# Autodesk Inventor assembly: robotModularAutoreconnfigurable
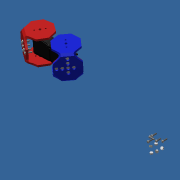
[picture p0: Inventor's stored thumbnail of the model, 180x180]
Saved by Autodesk Inventor 2014 (Build 180170000, 170)
## iProperties
Created: 2014-04-30
Part Number: robotModularAutoreconnfigurable
Document SubType Name: Assembly
Designer: Lefo
Author: Lefo
## Documents named in this file (9)
- C:\Users\Lefo\Documents\Inventor\academy\final project\robotModularAutoreconnfigurable.iam
- C:\Users\Lefo\Documents\Inventor\academy\servo power HD1501MG\servomotorFakeShast.iam
- C:\Users\Lefo\Documents\Inventor\academy\final project\linkoct.ipt
- C:\Users\Lefo\Documents\Inventor\academy\iman.ipt
- C:\Users\Lefo\Documents\Inventor\academy\portatuerca.ipt
- C:\Users\Lefo\Documents\Inventor\academy\final project\linkoctsecundario.ipt
- C:\Users\Lefo\Documents\Inventor\Content Center Files\R2014\en-US\ISO 7045(1)\ISO 7045 - M3 x 12 - 4.8 - HDIN EN ISO.ipt
- C:\Users\Lefo\Documents\Inventor\academy\servo power HD1501MG\acople para eje falso.ipt
- C:\Users\Lefo\Documents\Inventor\Content Center Files\R2014\en-US\ISO 7045(1)\ISO 7045 - M3 x 10 - 4.8 - HDIN EN ISO.ipt
## Components (30 placed, 8 different names)
1. servomotorFakeShast:1 [sub-assembly] — Mate:1, Flush:1, Flush:2, Insert:11, Insert:19
2. servomotorFakeShast:2 [sub-assembly] — Mate:1, Flush:1, Flush:2, Insert:10, Mate:2, Insert:18
3. linkoct:2 — Insert:3, Insert:4, Insert:5, Insert:6, Insert:7, Insert:8, Insert:9, Insert:11, Mate:3, Flush:3, Flush:4
4. iman:1 — Insert:3
5. portatuerca:1 — Mate:3, Flush:3, Flush:4
6. iman:2 — Insert:7
7. iman:3 — Insert:6
8. iman:4 — Insert:8
9. iman:5 — Insert:9
10. iman:6 — Insert:5
11. iman:7 — Insert:4
12. linkoctsecundario:1 — Insert:10, Mate:2, Insert:12, Insert:13, Insert:14, Insert:15, Insert:16, Insert:17
13. DIN EN ISO 7045 H M3 x 12 - 4.8 - H:1 — Insert:12
14. DIN EN ISO 7045 H M3 x 12 - 4.8 - H:2 — Insert:13
15. DIN EN ISO 7045 H M3 x 12 - 4.8 - H:3 — Insert:14
16. DIN EN ISO 7045 H M3 x 12 - 4.8 - H:4 — Insert:15
17. DIN EN ISO 7045 H M3 x 12 - 4.8 - H:5 — Insert:16
18. DIN EN ISO 7045 H M3 x 12 - 4.8 - H:6 — Insert:17
19. acople para eje falso:1 — Insert:19
20. acople para eje falso:2 — Insert:18
21. iman:8
22. iman:9
23. iman:10
24. iman:11
25. iman:12
26. DIN EN ISO 7045 H M3 x 10 - 4.8 - H:1
27. DIN EN ISO 7045 H M3 x 10 - 4.8 - H:2
28. DIN EN ISO 7045 H M3 x 10 - 4.8 - H:3
29. DIN EN ISO 7045 H M3 x 10 - 4.8 - H:4
30. DIN EN ISO 7045 H M3 x 10 - 4.8 - H:5
## Relationships (24: Insert 17, Flush 4, Mate 3)
- Mate:1: servomotorFakeShast:1 ↔ servomotorFakeShast:2
- Flush:1: servomotorFakeShast:1 ↔ servomotorFakeShast:2
- Flush:2: servomotorFakeShast:1 ↔ servomotorFakeShast:2
- Insert:3: linkoct:2 ↔ iman:1
- Insert:4: linkoct:2 ↔ iman:7
- Insert:5: linkoct:2 ↔ iman:6
- Insert:6: linkoct:2 ↔ iman:3
- Insert:7: linkoct:2 ↔ iman:2
- Insert:8: linkoct:2 ↔ iman:4
- Insert:9: linkoct:2 ↔ iman:5
- Insert:10: servomotorFakeShast:2 ↔ linkoctsecundario:1
- Mate:2: servomotorFakeShast:2 ↔ linkoctsecundario:1
- Insert:11: servomotorFakeShast:1 ↔ linkoct:2
- Insert:12: linkoctsecundario:1 ↔ DIN EN ISO 7045 H M3 x 12 - 4.8 - H:1
- Insert:13: linkoctsecundario:1 ↔ DIN EN ISO 7045 H M3 x 12 - 4.8 - H:2
- Insert:14: linkoctsecundario:1 ↔ DIN EN ISO 7045 H M3 x 12 - 4.8 - H:3
- Insert:15: linkoctsecundario:1 ↔ DIN EN ISO 7045 H M3 x 12 - 4.8 - H:4
- Insert:16: linkoctsecundario:1 ↔ DIN EN ISO 7045 H M3 x 12 - 4.8 - H:5
- Insert:17: linkoctsecundario:1 ↔ DIN EN ISO 7045 H M3 x 12 - 4.8 - H:6
- Insert:18: servomotorFakeShast:2 ↔ acople para eje falso:2
- Mate:3: linkoct:2 ↔ portatuerca:1
- Flush:3 (1 mm): linkoct:2 ↔ portatuerca:1
- Flush:4 (1 mm): linkoct:2 ↔ portatuerca:1
- Insert:19: servomotorFakeShast:1 ↔ acople para eje falso:1
